# Autodesk Inventor assembly: CascoV2
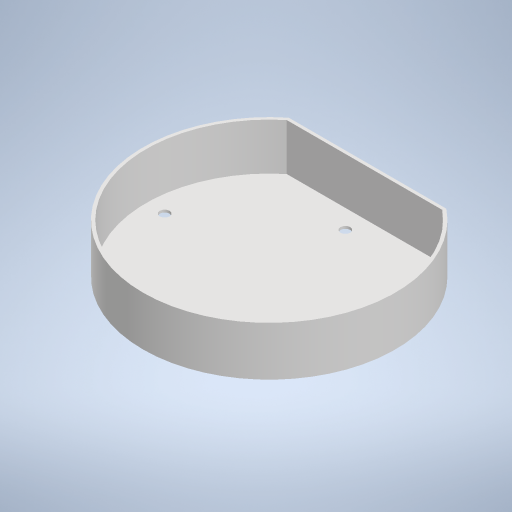
[picture p0: Inventor's stored thumbnail of the model, 512x512]
Saved by Autodesk Inventor 2024.2 (Build 282272000, 272)
## iProperties
Created: 2023-12-14
Part Number: CascoV2
Document SubType Name: Assembly
Designer: felip
Author: felip
## Documents named in this file (3)
- C:\Users\felip\OneDrive\Documentos\Robocupp-Mecanica\Gemelo Digital V2\CascoV2.iam
- C:\Users\felip\OneDrive\Documentos\Robocupp-Mecanica\Gemelo Digital V2\Casco.ipt
- C:\Users\felip\OneDrive\Documentos\Robocupp-Mecanica\Logo.ipt
## Components (2 placed, 2 different names)
1. Casco:1 — Mate:1
2. Logo:1 — Mate:1
## Relationships (1: Mate 1)
- Mate:1: Casco:1 ↔ Logo:1
